# Autodesk Inventor assembly: Sestava
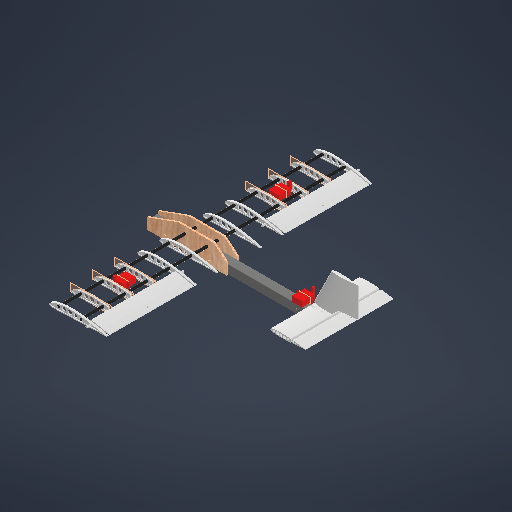
[picture p0: Inventor's stored thumbnail of the model, 512x512]
Saved by Autodesk Inventor 2026 (Build 300175050, 175E)
## iProperties
Created: 2026-02-21
Part Number: Sestava
Document SubType Name: Assembly
Designer: marti
Mass: 312.301 g
Surface Area: 1695.85 cm^2
Volume: 283.461 cm^3
Density: 1.10174 g/cm^3
Author: marti
## Documents named in this file (13)
- F:\Ročníkovka\RP_Svitek\3d model\lepší\Sestava.iam
- F:\Ročníkovka\RP_Svitek\3d model\lepší\tyč.ipt
- F:\Ročníkovka\RP_Svitek\3d model\lepší\Profil.ipt
- F:\Ročníkovka\RP_Svitek\3d model\lepší\NOAileron.ipt
- F:\Ročníkovka\RP_Svitek\3d model\lepší\Aileronn.ipt
- F:\Ročníkovka\RP_Svitek\3d model\lepší\vetrovaniig.ipt
- F:\Ročníkovka\RP_Svitek\3d model\lepší\Servo.ipt
- F:\Ročníkovka\RP_Svitek\3d model\lepší\Hlavni_pater.ipt
- F:\Ročníkovka\RP_Svitek\3d model\lepší\horizontal_stab.ipt
- F:\Ročníkovka\RP_Svitek\3d model\lepší\vertical_stab.ipt
- F:\Ročníkovka\RP_Svitek\3d model\lepší\horizontal_stab_elevator.ipt
- F:\Ročníkovka\RP_Svitek\3d model\lepší\Trup.ipt
- F:\Ročníkovka\RP_Svitek\3d model\lepší\motor držák.ipt
## Components (27 placed, 12 different names)
1. tyč:1 — Proti sobě:1, Stejný směr:1, Proti sobě:2, Proti sobě:3, Proti sobě:4, Proti sobě:8, Proti sobě:10, Proti sobě:12, Proti sobě:14, Proti sobě:17, Stejný směr:2, Proti sobě:22, Proti sobě:27, Proti sobě:29, Proti sobě:31, Proti sobě:56, Proti sobě:58, Proti sobě:75, Proti sobě:77, Stejný směr:20
2. tyč:2 — Proti sobě:4, Proti sobě:5, Proti sobě:6, Proti sobě:7, Proti sobě:9, Proti sobě:11, Proti sobě:13, Proti sobě:15, Proti sobě:18, Stejný směr:2, Stejný směr:3, Proti sobě:23, Stejný směr:4, Proti sobě:28, Proti sobě:30, Proti sobě:32, Proti sobě:57, Proti sobě:59, Proti sobě:76, Proti sobě:78
3. Profil:1 — Proti sobě:2, Proti sobě:6, Stejný směr:4, Proti sobě:24, Proti sobě:25, Stejný směr:5
4. Profil:2 — Proti sobě:3, Proti sobě:7, Proti sobě:16, Proti sobě:19, Proti sobě:20, Stejný směr:3, Stejný směr:9
5. NOAileron:1 — Proti sobě:8, Proti sobě:9, Stejný směr:5, Stejný směr:6
6. NOAileron:2 — Proti sobě:10, Proti sobě:11, Stejný směr:6, Stejný směr:7, Stejný směr:16
7. NOAileron:3 — Proti sobě:14, Proti sobě:15, Stejný směr:9, Stejný směr:10, Stejný směr:15
8. NOAileron:4 — Proti sobě:12, Proti sobě:13, Stejný směr:10, Stejný směr:11
9. Profil:3 — Proti sobě:22, Proti sobě:23, Proti sobě:26, Stejný směr:7, Stejný směr:8
10. Profil:4 — Proti sobě:17, Proti sobě:18, Proti sobě:21, Stejný směr:11, Stejný směr:12
11. Aileronn:1 — Proti sobě:16, Proti sobě:19, Proti sobě:20, Proti sobě:21
12. Aileronn:2 — Proti sobě:24, Proti sobě:25, Proti sobě:26
13. Profil:5 — Proti sobě:27, Proti sobě:28, Stejný směr:8, Stejný směr:17
14. Profil:6 — Proti sobě:29, Proti sobě:30, Stejný směr:12, Stejný směr:13
15. vetrovaniig:1 — Proti sobě:31, Proti sobě:32, Stejný směr:13
16. Servo:1
17. Servo:2
18. NOAileron:5 — Proti sobě:56, Proti sobě:57, Stejný směr:15
19. NOAileron:6 — Proti sobě:58, Proti sobě:59, Stejný směr:16
20. Hlavni_pater:1 — Proti sobě:67, Proti sobě:68, Proti sobě:69, Proti sobě:74, Stejný směr:18, Proti sobě:79, Proti sobě:80, Stejný směr:19, Stejný směr:20, Proti sobě:85, Proti sobě:86, Proti sobě:87
21. horizontal_stab:1 — Proti sobě:67, Proti sobě:68, Proti sobě:69, Proti sobě:71, Proti sobě:72, Proti sobě:73, Stejný směr:17, Proti sobě:81, Proti sobě:82, Proti sobě:88, Proti sobě:89, Proti sobě:90
22. Servo:3 — Proti sobě:74, Stejný směr:18
23. vertical_stab:1 — Proti sobě:71, Proti sobě:72, Proti sobě:73, Proti sobě:88, Proti sobě:89, Proti sobě:90
24. horizontal_stab_elevator:1 — Proti sobě:81, Proti sobě:82
25. Trup:1 — Proti sobě:75, Proti sobě:76, Proti sobě:79, Stejný směr:19
26. Trup:2 — Proti sobě:77, Proti sobě:78, Proti sobě:80
27. motor držák:1 — Proti sobě:85, Proti sobě:86, Proti sobě:87
## Relationships (76: Mate 57, Flush 19)
- Proti sobě:1 [Mate]: tyč:1
- Stejný směr:1 [Flush]: tyč:1
- Proti sobě:2 [Mate]: tyč:1 ↔ Profil:1
- Proti sobě:3 [Mate]: tyč:1 ↔ Profil:2
- Proti sobě:4 [Mate] (-50 mm): tyč:1 ↔ tyč:2
- Proti sobě:5 [Mate]: tyč:2
- Proti sobě:6 [Mate]: tyč:2 ↔ Profil:1
- Proti sobě:7 [Mate]: tyč:2 ↔ Profil:2
- Proti sobě:8 [Mate]: tyč:1 ↔ NOAileron:1
- Proti sobě:9 [Mate]: tyč:2 ↔ NOAileron:1
- Proti sobě:10 [Mate]: tyč:1 ↔ NOAileron:2
- Proti sobě:11 [Mate]: tyč:2 ↔ NOAileron:2
- Proti sobě:12 [Mate]: tyč:1 ↔ NOAileron:4
- Proti sobě:13 [Mate]: tyč:2 ↔ NOAileron:4
- Proti sobě:14 [Mate]: tyč:1 ↔ NOAileron:3
- Proti sobě:15 [Mate]: tyč:2 ↔ NOAileron:3
- Proti sobě:16 [Mate]: Profil:2 ↔ Aileronn:1
- Proti sobě:17 [Mate]: tyč:1 ↔ Profil:4
- Proti sobě:18 [Mate]: tyč:2 ↔ Profil:4
- Proti sobě:19 [Mate]: Profil:2 ↔ Aileronn:1
- Proti sobě:20 [Mate] (2 mm): Profil:2 ↔ Aileronn:1
- Stejný směr:2 [Flush]: tyč:1 ↔ tyč:2
- Stejný směr:3 [Flush]: tyč:2 ↔ Profil:2
- Proti sobě:21 [Mate] (2 mm): Profil:4 ↔ Aileronn:1
- Proti sobě:22 [Mate]: tyč:1 ↔ Profil:3
- Proti sobě:23 [Mate]: tyč:2 ↔ Profil:3
- Stejný směr:4 [Flush]: tyč:2 ↔ Profil:1
- Proti sobě:24 [Mate]: Profil:1 ↔ Aileronn:2
- Proti sobě:25 [Mate] (2 mm): Profil:1 ↔ Aileronn:2
- Proti sobě:26 [Mate] (2 mm): Profil:3 ↔ Aileronn:2
- Proti sobě:27 [Mate]: tyč:1 ↔ Profil:5
- Proti sobě:28 [Mate]: tyč:2 ↔ Profil:5
- Proti sobě:29 [Mate]: tyč:1 ↔ Profil:6
- Proti sobě:30 [Mate]: tyč:2 ↔ Profil:6
- Stejný směr:5 [Flush] (50 mm): Profil:1 ↔ NOAileron:1
- Stejný směr:6 [Flush] (-100 mm): NOAileron:1 ↔ NOAileron:2
- Stejný směr:7 [Flush] (-50 mm): NOAileron:2 ↔ Profil:3
- Stejný směr:8 [Flush] (50 mm): Profil:3 ↔ Profil:5
- Stejný směr:9 [Flush] (50 mm): Profil:2 ↔ NOAileron:3
- Stejný směr:10 [Flush] (100 mm): NOAileron:3 ↔ NOAileron:4
- Stejný směr:11 [Flush] (50 mm): NOAileron:4 ↔ Profil:4
- Stejný směr:12 [Flush] (50 mm): Profil:4 ↔ Profil:6
- Proti sobě:31 [Mate]: tyč:1 ↔ vetrovaniig:1
- Proti sobě:32 [Mate]: tyč:2 ↔ vetrovaniig:1
- Stejný směr:13 [Flush] (-48 mm): Profil:6 ↔ vetrovaniig:1
- Proti sobě:56 [Mate]: tyč:1 ↔ NOAileron:5
- Proti sobě:57 [Mate]: tyč:2 ↔ NOAileron:5
- Stejný směr:15 [Flush] (50 mm): NOAileron:3 ↔ NOAileron:5
- Proti sobě:58 [Mate]: tyč:1 ↔ NOAileron:6
- Proti sobě:59 [Mate]: tyč:2 ↔ NOAileron:6
- Stejný směr:16 [Flush] (50 mm): NOAileron:2 ↔ NOAileron:6
- Proti sobě:67 [Mate]: Hlavni_pater:1 ↔ horizontal_stab:1
- Proti sobě:68 [Mate]: Hlavni_pater:1 ↔ horizontal_stab:1
- Proti sobě:69 [Mate]: Hlavni_pater:1 ↔ horizontal_stab:1
- Proti sobě:71 [Mate]: horizontal_stab:1 ↔ vertical_stab:1
- Proti sobě:72 [Mate]: horizontal_stab:1 ↔ vertical_stab:1
- Proti sobě:73 [Mate]: horizontal_stab:1 ↔ vertical_stab:1
- Stejný směr:17 [Flush] (300 mm): Profil:5 ↔ horizontal_stab:1
- Proti sobě:74 [Mate]: Hlavni_pater:1 ↔ Servo:3
- Stejný směr:18 [Flush] (-7.5 mm): Hlavni_pater:1 ↔ Servo:3
- Proti sobě:75 [Mate]: tyč:1 ↔ Trup:1
- Proti sobě:76 [Mate]: tyč:2 ↔ Trup:1
- Proti sobě:77 [Mate]: tyč:1 ↔ Trup:2
- Proti sobě:78 [Mate]: tyč:2 ↔ Trup:2
- Proti sobě:79 [Mate]: Hlavni_pater:1 ↔ Trup:1
- Proti sobě:80 [Mate]: Hlavni_pater:1 ↔ Trup:2
- Stejný směr:19 [Flush]: Hlavni_pater:1 ↔ Trup:1
- Proti sobě:81 [Mate]: horizontal_stab:1 ↔ horizontal_stab_elevator:1
- Proti sobě:82 [Mate]: horizontal_stab:1 ↔ horizontal_stab_elevator:1
- Stejný směr:20 [Flush] (300 mm): tyč:1 ↔ Hlavni_pater:1
- Proti sobě:85 [Mate]: Hlavni_pater:1 ↔ motor držák:1
- Proti sobě:86 [Mate]: Hlavni_pater:1 ↔ motor držák:1
- Proti sobě:87 [Mate]: Hlavni_pater:1 ↔ motor držák:1
- Proti sobě:88 [Mate]: horizontal_stab:1 ↔ vertical_stab:1
- Proti sobě:89 [Mate]: horizontal_stab:1 ↔ vertical_stab:1
- Proti sobě:90 [Mate]: horizontal_stab:1 ↔ vertical_stab:1
